# Autodesk Inventor assembly: Gripper6
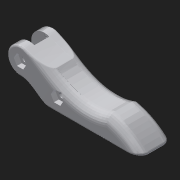
[picture p0: Inventor's stored thumbnail of the model, 180x180]
Saved by Autodesk Inventor 2017 SP1 (Build 210196100, 196)
## iProperties
Created: 2018-03-03
Part Number: Gripper6
Document SubType Name: Assembly
Designer: Zach
Author: Zach
## Documents named in this file (2)
- C:\Users\Zach\Documents\GitHub\tr1_description\meshes\Visual Assembly\Gripper6.iam
- C:\Users\Zach\Desktop\gripper6.ipt
## Components (1 placed, 1 different names)
1. gripper6:1 — Mate:1, Angle:1, Mate:2
## Relationships (3: Mate 2, Angle 1)
- Mate:1: gripper6:1
- Angle:1 (180 deg): gripper6:1
- Mate:2 (4 mm): gripper6:1
